# Autodesk Inventor assembly: leg
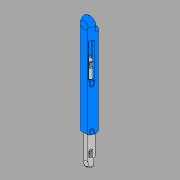
[picture p0: Inventor's stored thumbnail of the model, 180x180]
Saved by Autodesk Inventor 2020 (Build 240168000, 168)
## iProperties
Created: 2020-12-28
Part Number: leg
Document SubType Name: Assembly
Designer: freyja
Author: freyja
## Documents named in this file (3)
- C:\Users\freyja\Documents\OpenSpace\CAD\leg.iam
- C:\Users\freyja\Documents\OpenSpace\CAD\inner leg.ipt
- C:\Users\freyja\Documents\OpenSpace\CAD\outer leg.ipt
## Components (2 placed, 2 different names)
1. inner leg:1 — Mate:1
2. outer leg:1 — Mate:1, Angle:1
## Relationships (2: Mate 1, Angle 1)
- Mate:1: inner leg:1 ↔ outer leg:1
- Angle:1 (0 deg): outer leg:1
